# Autodesk Inventor assembly: Boitier_Phoenix_A150
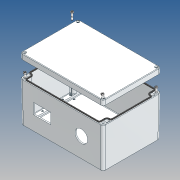
[picture p0: Inventor's stored thumbnail of the model, 180x180]
Saved by Autodesk Inventor 2021.3 (Build 253353000, 353)
## iProperties
Company: Ifina
Created: 2021-11-11
Part Number: Boitier_Phoenix_A150
Description: STEP AP214
Document SubType Name: Assembly
Designer: gabri
Sending System: SolidWorks 2020
Preprocessor: SwSTEP 2.0
Title: 01233318.STEP
Author: Ifina
Revision Number: ANY
## Documents named in this file (5)
- D:\PGA\Boitier_Phoenix_A150.iam
- D:\PGA\01621_01-2-016210-01-0.ipt
- D:\PGA\02062_Bearbeitung n. Zeichn. (01-2-021510-03-0).ipt
- D:\PGA\93134.ipt
- D:\PGA\99999_1040_Fr Deckel 02062.ipt
## Components (7 placed, 7 different names)
1. 01621_01-2-016210-01-0_1 — Mate:1, Mate:2
2. 02062_Bearbeitung n. Zeichn. (01-2-021510-03-0)_2 — Mate:1, Mate:2
3. 93134_3
4. 93134_4
5. 93134_5
6. 93134_6
7. 99999_1040_Fr Deckel 02062_7
## Relationships (2: Mate 2)
- Mate:1: 01621_01-2-016210-01-0_1 ↔ 02062_Bearbeitung n. Zeichn. (01-2-021510-03-0)_2
- Mate:2: 01621_01-2-016210-01-0_1 ↔ 02062_Bearbeitung n. Zeichn. (01-2-021510-03-0)_2
